# Autodesk Inventor assembly: Assembly1
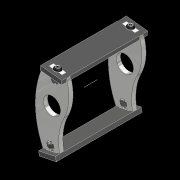
[picture p0: Inventor's stored thumbnail of the model, 180x180]
Saved by Autodesk Inventor 2022 (Build 260153000, 153)
## iProperties
Created: 2023-01-22
Part Number: Assembly1
Document SubType Name: Assembly
Designer: tandu
Mass: 312.879 g
Surface Area: 345.322 cm^2
Volume: 70.4332 cm^3
Author: tandu
## Documents named in this file (7)
- C:\Users\tandu\Documents\GrabCAD\CustomBeaterBar\3lb\WDTooth\Assembly1.iam
- C:\Users\tandu\Documents\GrabCAD\CustomBeaterBar\3lb\WDTooth\Parameter Part CBB.ipt
- C:\Users\tandu\Documents\GrabCAD\CustomBeaterBar\3lb\WDTooth\Bar.ipt
- C:\Users\tandu\Documents\GrabCAD\CustomBeaterBar\3lb\WDTooth\Impactor.ipt
- C:\Users\tandu\Documents\GrabCAD\CustomBeaterBar\3lb\WDTooth\94166A130_Black-Oxide High-Strength steel Hex nut.ipt
- C:\Users\tandu\Documents\GrabCAD\CustomBeaterBar\3lb\WDTooth\91239A323_Button Head Hex Drive Screw.ipt
- C:\Users\tandu\Documents\GrabCAD\CustomBeaterBar\3lb\WDTooth\CW.ipt
## Components (13 placed, 6 different names)
1. Parameter Part CBB:1
2. Bar:1 — Mate:1, Angle:1, Mate:3, Mate:4, Mate:5, Symmetry:1, Mate:8, Mate:9, Mate:15, Mate:24, Mate:25, Mate:26, Mate:27, Mate:28, Mate:29
3. Bar:2 — Mate:2, Angle:1, Mate:6, Symmetry:1, Mate:16, Mate:17, Mate:21, Mate:30, Mate:31, Mate:32
4. Impactor:1 — Mate:3, Mate:4, Mate:5, Mate:6, Mate:11, Mate:23
5. CW:1 — Mate:24, Mate:25, Mate:26, Mate:34, Mate:36
6. 94166A130_Black-Oxide High-Strength steel Hex nut:1 — Mate:8, Mate:9, Mate:10, Mate:12, Mate:13, Mate:14
7. 94166A130_Black-Oxide High-Strength steel Hex nut:2 — Mate:16, Mate:17, Mate:18, Mate:19, Mate:20, Mate:22
8. 94166A130_Black-Oxide High-Strength steel Hex nut:3 — Mate:27, Mate:28, Mate:29, Mate:33
9. 94166A130_Black-Oxide High-Strength steel Hex nut:4 — Mate:30, Mate:31, Mate:32, Mate:35
10. 91239A323_Button Head Hex Drive Screw:1 — Mate:10, Mate:11
11. 91239A323_Button Head Hex Drive Screw:2 — Mate:22, Mate:23
12. 91239A323_Button Head Hex Drive Screw:3 — Mate:33, Mate:34
13. 91239A323_Button Head Hex Drive Screw:4 — Mate:35, Mate:36
## Relationships (38: Mate 36, Angle 1, Symmetry 1)
- Mate:1: Bar:1
- Mate:2: Bar:2
- Angle:1 (0 deg): Bar:1 ↔ Bar:2
- Mate:3: Bar:1 ↔ Impactor:1
- Mate:4: Bar:1 ↔ Impactor:1
- Mate:5: Bar:1 ↔ Impactor:1
- Mate:6: Bar:2 ↔ Impactor:1
- Symmetry:1: Bar:1 ↔ Bar:2
- Mate:7
- Mate:8: Bar:1 ↔ 94166A130_Black-Oxide High-Strength steel Hex nut:1
- Mate:9: Bar:1 ↔ 94166A130_Black-Oxide High-Strength steel Hex nut:1
- Mate:10: 94166A130_Black-Oxide High-Strength steel Hex nut:1 ↔ 91239A323_Button Head Hex Drive Screw:1
- Mate:11: Impactor:1 ↔ 91239A323_Button Head Hex Drive Screw:1
- Mate:12: 94166A130_Black-Oxide High-Strength steel Hex nut:1
- Mate:13: 94166A130_Black-Oxide High-Strength steel Hex nut:1
- Mate:14: 94166A130_Black-Oxide High-Strength steel Hex nut:1
- Mate:15: Bar:1
- Mate:16: Bar:2 ↔ 94166A130_Black-Oxide High-Strength steel Hex nut:2
- Mate:17: Bar:2 ↔ 94166A130_Black-Oxide High-Strength steel Hex nut:2
- Mate:18: 94166A130_Black-Oxide High-Strength steel Hex nut:2
- Mate:19: 94166A130_Black-Oxide High-Strength steel Hex nut:2
- Mate:20: 94166A130_Black-Oxide High-Strength steel Hex nut:2
- Mate:21: Bar:2
- Mate:22: 94166A130_Black-Oxide High-Strength steel Hex nut:2 ↔ 91239A323_Button Head Hex Drive Screw:2
- Mate:23: Impactor:1 ↔ 91239A323_Button Head Hex Drive Screw:2
- Mate:24: Bar:1 ↔ CW:1
- Mate:25: Bar:1 ↔ CW:1
- Mate:26: Bar:1 ↔ CW:1
- Mate:27: Bar:1 ↔ 94166A130_Black-Oxide High-Strength steel Hex nut:3
- Mate:28: Bar:1 ↔ 94166A130_Black-Oxide High-Strength steel Hex nut:3
- Mate:29: Bar:1 ↔ 94166A130_Black-Oxide High-Strength steel Hex nut:3
- Mate:30: Bar:2 ↔ 94166A130_Black-Oxide High-Strength steel Hex nut:4
- Mate:31: Bar:2 ↔ 94166A130_Black-Oxide High-Strength steel Hex nut:4
- Mate:32: Bar:2 ↔ 94166A130_Black-Oxide High-Strength steel Hex nut:4
- Mate:33: 94166A130_Black-Oxide High-Strength steel Hex nut:3 ↔ 91239A323_Button Head Hex Drive Screw:3
- Mate:34: CW:1 ↔ 91239A323_Button Head Hex Drive Screw:3
- Mate:35: 94166A130_Black-Oxide High-Strength steel Hex nut:4 ↔ 91239A323_Button Head Hex Drive Screw:4
- Mate:36: CW:1 ↔ 91239A323_Button Head Hex Drive Screw:4
